# Autodesk Inventor assembly: HeadSlider
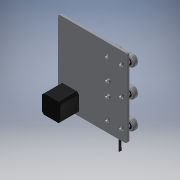
[picture p0: Inventor's stored thumbnail of the model, 180x180]
Saved by Autodesk Inventor 2017 (Build 210142000, 142)
## iProperties
Created: 2016-12-13
Part Number: HeadSlider
Document SubType Name: Assembly
Designer: umr
Author: umr
## Documents named in this file (6)
- D:\SeniorProject\Models2\Head\HeadSlider.iam
- D:\SeniorProject\Models2\Head\HeadPlate.ipt
- D:\SeniorProject\Models2\Head\Solid Wheel with Eccentric Spacer Assembly.iam
- D:\SeniorProject\Models2\Head\Motor.ipt
- D:\SeniorProject\Models2\Head\GT2 20 Tooth Pulley.ipt
- D:\SeniorProject\Models2\Head\HeaderSliderBelt.ipt
## Components (11 placed, 5 different names)
1. HeadPlate:1 — Mate:1, Mate:2, Mate:3, Mate:4, Mate:5, Mate:6, Mate:7, Mate:8, Mate:9, Mate:10, Mate:11, Mate:12, Mate:13, Mate:14, Mate:15, Mate:16, Mate:17, Mate:18, Mate:20
2. Solid Wheel with Eccentric Spacer Assembly:1 [sub-assembly] — Mate:3, Mate:8
3. Solid Wheel with Eccentric Spacer Assembly:2 [sub-assembly] — Mate:4, Mate:9, Tangent:1
4. Solid Wheel with Eccentric Spacer Assembly:3 [sub-assembly] — Mate:6, Mate:11
5. Solid Wheel with Eccentric Spacer Assembly:4 [sub-assembly] — Mate:1, Mate:13
6. Solid Wheel with Eccentric Spacer Assembly:5 [sub-assembly] — Mate:2, Mate:14
7. Solid Wheel with Eccentric Spacer Assembly:6 [sub-assembly] — Mate:5, Mate:12
8. Solid Wheel with Eccentric Spacer Assembly:7 [sub-assembly] — Mate:7, Mate:10, Tangent:2
9. Motor:1 — Mate:15, Mate:16, Mate:17, Mate:18, Mate:19
10. GT2 20 Tooth Pulley:1 — Mate:19, Mate:20
11. HeaderSliderBelt:1 — Tangent:1, Tangent:2
## Relationships (22: Mate 20, Tangent 2)
- Mate:1: HeadPlate:1 ↔ Solid Wheel with Eccentric Spacer Assembly:4
- Mate:2: HeadPlate:1 ↔ Solid Wheel with Eccentric Spacer Assembly:5
- Mate:3: HeadPlate:1 ↔ Solid Wheel with Eccentric Spacer Assembly:1
- Mate:4: HeadPlate:1 ↔ Solid Wheel with Eccentric Spacer Assembly:2
- Mate:5: HeadPlate:1 ↔ Solid Wheel with Eccentric Spacer Assembly:6
- Mate:6: HeadPlate:1 ↔ Solid Wheel with Eccentric Spacer Assembly:3
- Mate:7: HeadPlate:1 ↔ Solid Wheel with Eccentric Spacer Assembly:7
- Mate:8: HeadPlate:1 ↔ Solid Wheel with Eccentric Spacer Assembly:1
- Mate:9: HeadPlate:1 ↔ Solid Wheel with Eccentric Spacer Assembly:2
- Mate:10: HeadPlate:1 ↔ Solid Wheel with Eccentric Spacer Assembly:7
- Mate:11: HeadPlate:1 ↔ Solid Wheel with Eccentric Spacer Assembly:3
- Mate:12: HeadPlate:1 ↔ Solid Wheel with Eccentric Spacer Assembly:6
- Mate:13: HeadPlate:1 ↔ Solid Wheel with Eccentric Spacer Assembly:4
- Mate:14: HeadPlate:1 ↔ Solid Wheel with Eccentric Spacer Assembly:5
- Mate:15: HeadPlate:1 ↔ Motor:1
- Mate:16: HeadPlate:1 ↔ Motor:1
- Mate:17: HeadPlate:1 ↔ Motor:1
- Mate:18: HeadPlate:1 ↔ Motor:1
- Mate:19: Motor:1 ↔ GT2 20 Tooth Pulley:1
- Mate:20: HeadPlate:1 ↔ GT2 20 Tooth Pulley:1
- Tangent:1: Solid Wheel with Eccentric Spacer Assembly:2 ↔ HeaderSliderBelt:1
- Tangent:2: Solid Wheel with Eccentric Spacer Assembly:7 ↔ HeaderSliderBelt:1
